# Autodesk Inventor assembly: R2_オムニ
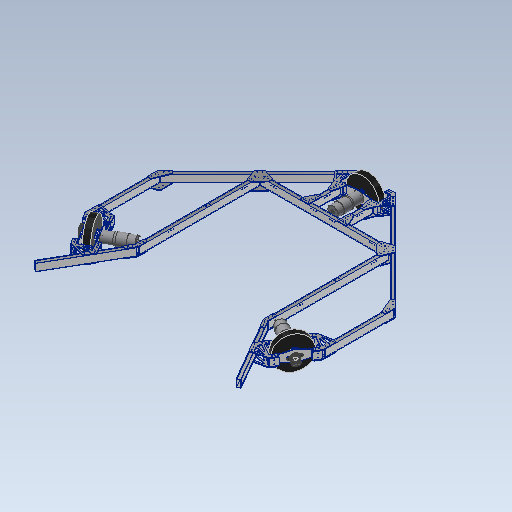
[picture p0: Inventor's stored thumbnail of the model, 512x512]
Saved by Autodesk Inventor 2021 (Build 250183000, 183)
## iProperties
Created: 2021-12-02
Part Number: R2_オムニ
Material: 一般
Document SubType Name: Assembly
Designer: 堀川皓史
Mass: 8176.66 g
Surface Area: 23070.1 cm^2
Volume: 4150.36 cm^3
Density: 1.97011 g/cm^3
Author: 堀川皓史
## Documents named in this file (23)
- C:\Users\hirohumi\OneDrive\ドキュメント\ロボ研\2022NHKロボコン\R2_version1\R2_オムニ.iam
- C:\Users\hirohumi\OneDrive\ドキュメント\ロボ研\2022NHKロボコン\オムニホイール\角柱40mm_モータエンコーダ固定用.ipt
- C:\Users\hirohumi\OneDrive\ドキュメント\ロボ研\2022NHKロボコン\オムニホイール\ホイールユニット_モータ固定板.ipt
- C:\Users\hirohumi\OneDrive\ドキュメント\ロボ研\2022NHKロボコン\オムニホイール\RS-775GM017 v1.ipt
- C:\Users\hirohumi\OneDrive\ドキュメント\ロボ研\2022NHKロボコン\オムニホイール\ホイールユニット_エンコーダ取付板.ipt
- C:\Users\hirohumi\OneDrive\ドキュメント\ロボ研\2022NHKロボコン\オムニホイール\amt102-v v3\amt102-v.iam
- C:\Users\hirohumi\OneDrive\ドキュメント\ロボ研\2022NHKロボコン\オムニホイール\オムニホイール_8-135.ipt
- C:\Users\hirohumi\OneDrive\ドキュメント\ロボ研\2022NHKロボコン\オムニホイール\オムニ固定する.ipt
- C:\Users\hirohumi\OneDrive\ドキュメント\ロボ研\2022NHKロボコン\R2_version1\オムニ_後ろ側板.ipt
- C:\Users\hirohumi\OneDrive\ドキュメント\ロボ研\2022NHKロボコン\R2_version1\オムニ_前1側板.ipt
- C:\Users\hirohumi\OneDrive\ドキュメント\ロボ研\2022NHKロボコン\R2_version1\オムニ_前2側板.ipt
- C:\Users\hirohumi\OneDrive\ドキュメント\ロボ研\2022NHKロボコン\R2_version1\オムニ_角柱1.ipt
- C:\Users\hirohumi\OneDrive\ドキュメント\ロボ研\2022NHKロボコン\オムニホイール\角柱40mm_モータエンコーダ固定用小.ipt
- C:\Users\hirohumi\OneDrive\ドキュメント\ロボ研\2022NHKロボコン\R2_version1\オムニ_固定具1.ipt
- C:\Users\hirohumi\OneDrive\ドキュメント\ロボ研\2022NHKロボコン\R2_version1\オムニ_角柱2.ipt
- C:\Users\hirohumi\OneDrive\ドキュメント\ロボ研\2022NHKロボコン\R2_version1\オムニ_角柱5.ipt
- C:\Users\hirohumi\OneDrive\ドキュメント\ロボ研\2022NHKロボコン\R2_version1\オムニ_固定具2.ipt
- C:\Users\hirohumi\OneDrive\ドキュメント\ロボ研\2022NHKロボコン\R2_version1\オムニ_角柱3.ipt
- C:\Users\hirohumi\OneDrive\ドキュメント\ロボ研\2022NHKロボコン\R2_version1\オムニ_角柱4.ipt
- C:\Users\hirohumi\OneDrive\ドキュメント\ロボ研\2022NHKロボコン\R2_version1\オムニ_固定具3.ipt
- C:\Users\hirohumi\OneDrive\ドキュメント\ロボ研\2022NHKロボコン\R2_version1\オムニ_固定具1-1.ipt
- C:\Users\hirohumi\OneDrive\ドキュメント\ロボ研\2022NHKロボコン\R2_version1\オムニ_角柱7.ipt
- C:\Users\hirohumi\OneDrive\ドキュメント\ロボ研\2022NHKロボコン\R2_version1\オムニ_koteigu.ipt
## Components (70 placed, 22 different names)
1. 角柱40mm_モータエンコーダ固定用:1 — 挿入:17, 挿入:18, 挿入:19
2. 角柱40mm_モータエンコーダ固定用:3 — 挿入:21, 挿入:23
3. ホイールユニット_モータ固定板:1
4. RS-775GM017 v1:1
5. ホイールユニット_エンコーダ取付板:1
6. amt102-v:1 [sub-assembly]
7. オムニホイール_8-135:1
8. オムニ固定する:1
9. オムニ固定する:2
10. オムニ_後ろ側板:1 — 挿入:17, 挿入:18, 挿入:77, 挿入:78, 挿入:81, 挿入:82, 挿入:184, 挿入:185
11. オムニ_後ろ側板:2 — 挿入:19
12. オムニ_後ろ側板:3 — 挿入:21
13. オムニ_後ろ側板:4 — 挿入:23, 挿入:79, 挿入:80, 挿入:83, 挿入:84, 挿入:182, 挿入:183
14. 角柱40mm_モータエンコーダ固定用:5 — 挿入:48, 挿入:50, 挿入:111
15. 角柱40mm_モータエンコーダ固定用:7 — 挿入:41, 挿入:42, 挿入:45, 挿入:112
16. ホイールユニット_モータ固定板:2
17. RS-775GM017 v1:2
18. ホイールユニット_エンコーダ取付板:2 — 挿入:95, 挿入:96
19. amt102-v:2 [sub-assembly]
20. オムニホイール_8-135:2
21. オムニ固定する:3
22. オムニ固定する:4
23. オムニ_前2側板:1 — 挿入:41, 挿入:42, 挿入:87, 挿入:88, 挿入:118, 挿入:119
24. オムニ_前2側板:2 — 挿入:45, 挿入:112
25. オムニ_前1側板:1 — 挿入:50, 挿入:85, 挿入:86, 挿入:109, 挿入:110, 挿入:111
26. オムニ_前1側板:2 — 挿入:48, 挿入:150
27. 角柱40mm_モータエンコーダ固定用:9 — 挿入:115, 挿入:116
28. 角柱40mm_モータエンコーダ固定用:11 — 挿入:117
29. ホイールユニット_モータ固定板:3
30. RS-775GM017 v1:3
31. ホイールユニット_エンコーダ取付板:3 — 挿入:93, 挿入:94
32. amt102-v:3 [sub-assembly]
33. オムニホイール_8-135:3
34. オムニ固定する:5
35. オムニ固定する:6
36. オムニ_前2側板:3 — 挿入:91, 挿入:92
37. オムニ_前2側板:4 — 挿入:117, 挿入:120, 挿入:121
38. オムニ_前1側板:3 — 挿入:89, 挿入:90, 挿入:113, 挿入:114, 挿入:116
39. オムニ_前1側板:4 — 挿入:115
40. オムニ_角柱1:1 — 挿入:77, 挿入:78, 挿入:134, 挿入:135, 挿入:144, 挿入:165, 挿入:167
41. オムニ_角柱1:2 — 挿入:79, 挿入:80, 挿入:140, 挿入:141, 挿入:147, 挿入:178, 挿入:181
42. 角柱40mm_モータエンコーダ固定用小:1 — 挿入:81, 挿入:82
43. 角柱40mm_モータエンコーダ固定用小:2 — 挿入:83, 挿入:84
44. 角柱40mm_モータエンコーダ固定用小:3 — 挿入:89, 挿入:90
45. 角柱40mm_モータエンコーダ固定用小:4 — 挿入:85, 挿入:86, 挿入:150
46. 角柱40mm_モータエンコーダ固定用小:5 — 挿入:91, 挿入:92, 挿入:93, 挿入:94
47. 角柱40mm_モータエンコーダ固定用小:6 — 挿入:87, 挿入:88, 挿入:95, 挿入:96
48. オムニ_固定具1:1 — 挿入:164, 挿入:165
49. オムニ_固定具1:2 — 挿入:177, 挿入:178, 挿入:179
50. オムニ_角柱2:1 — 挿入:109, 挿入:110, 挿入:164, 挿入:166
51. オムニ_角柱2:2 — 挿入:113, 挿入:114, 挿入:177, 挿入:179, 挿入:180
52. オムニ_角柱5:1 — 挿入:118, 挿入:119, 挿入:122, 挿入:123, 挿入:124, 挿入:125
53. オムニ_角柱5:2 — 挿入:120, 挿入:121, 挿入:126, 挿入:127, 挿入:128, 挿入:129
54. オムニ_固定具2:1 — 挿入:122, 挿入:123, 挿入:130, 挿入:131
55. オムニ_固定具2:2 — 挿入:124, 挿入:125
56. オムニ_固定具2:3 — 挿入:128, 挿入:129, 挿入:132, 挿入:133
57. オムニ_固定具2:4 — 挿入:126, 挿入:127
58. オムニ_角柱3:1 — 挿入:130, 挿入:131, 挿入:136, 挿入:137, 挿入:145
59. オムニ_角柱3:2 — 挿入:132, 挿入:133, 挿入:143, 挿入:148
60. オムニ_角柱4:1 — 挿入:138, 挿入:139, 挿入:142, 挿入:146, 挿入:149, フラッシュ:1, フラッシュ:2, 挿入:186
61. オムニ_固定具3:1 — 挿入:134, 挿入:135, 挿入:136, 挿入:137, 挿入:138, 挿入:139
62. オムニ_固定具3:2 — 挿入:147, 挿入:148, 挿入:149
63. オムニ_固定具3:3 — 挿入:144, 挿入:145, 挿入:146
64. オムニ_固定具3:4 — 挿入:140, 挿入:141, 挿入:142, 挿入:143
65. オムニ_固定具1-1:1 — 挿入:180, 挿入:181
66. オムニ_固定具1-1:2 — 挿入:166, 挿入:167
67. オムニ_角柱7:1 — 挿入:182, 挿入:183, 挿入:187
68. オムニ_角柱7:2 — 挿入:184, 挿入:185
69. オムニ_koteigu:1 — フラッシュ:1, フラッシュ:2
70. オムニ_koteigu:2 — 挿入:186, 挿入:187
## Relationships (133: Insert 125, Mate 6, Flush 2)
- [Insert]: 角柱40mm_モータエンコーダ固定用:1 ↔ ホイールユニット_モータ固定板:1
- [Insert]: 角柱40mm_モータエンコーダ固定用:1 ↔ ホイールユニット_モータ固定板:1
- [Insert]: 角柱40mm_モータエンコーダ固定用:3 ↔ ホイールユニット_モータ固定板:1
- [Insert]: 角柱40mm_モータエンコーダ固定用:3 ↔ ホイールユニット_モータ固定板:1
- [Insert]: ホイールユニット_モータ固定板:1 ↔ RS-775GM017 v1:1
- [Insert]: ホイールユニット_モータ固定板:1 ↔ RS-775GM017 v1:1
- [Insert]: ホイールユニット_エンコーダ取付板:1 ↔ amt102-v:1
- [Insert]: オムニホイール_8-135:1 ↔ オムニ固定する:1
- [Insert]: オムニホイール_8-135:1 ↔ オムニ固定する:1
- [Insert]: オムニホイール_8-135:1 ↔ オムニ固定する:2
- [Insert]: オムニホイール_8-135:1 ↔ オムニ固定する:2
- [Mate]: RS-775GM017 v1:1 ↔ オムニ固定する:1
- [Mate] (6 mm): ホイールユニット_モータ固定板:1 ↔ オムニ固定する:1
- 挿入:17 [Insert]: 角柱40mm_モータエンコーダ固定用:1 ↔ オムニ_後ろ側板:1
- 挿入:18 [Insert]: 角柱40mm_モータエンコーダ固定用:1 ↔ オムニ_後ろ側板:1
- 挿入:19 [Insert]: 角柱40mm_モータエンコーダ固定用:1 ↔ オムニ_後ろ側板:2
- 挿入:21 [Insert]: 角柱40mm_モータエンコーダ固定用:3 ↔ オムニ_後ろ側板:3
- 挿入:23 [Insert]: 角柱40mm_モータエンコーダ固定用:3 ↔ オムニ_後ろ側板:4
- [Insert]: 角柱40mm_モータエンコーダ固定用:5 ↔ ホイールユニット_モータ固定板:2
- [Insert]: 角柱40mm_モータエンコーダ固定用:5 ↔ ホイールユニット_モータ固定板:2
- [Insert]: 角柱40mm_モータエンコーダ固定用:7 ↔ ホイールユニット_モータ固定板:2
- [Insert]: 角柱40mm_モータエンコーダ固定用:7 ↔ ホイールユニット_モータ固定板:2
- [Insert]: ホイールユニット_モータ固定板:2 ↔ RS-775GM017 v1:2
- [Insert]: ホイールユニット_モータ固定板:2 ↔ RS-775GM017 v1:2
- [Insert]: ホイールユニット_エンコーダ取付板:2 ↔ amt102-v:2
- [Insert]: オムニホイール_8-135:2 ↔ オムニ固定する:3
- [Insert]: オムニホイール_8-135:2 ↔ オムニ固定する:3
- [Insert]: オムニホイール_8-135:2 ↔ オムニ固定する:4
- [Insert]: オムニホイール_8-135:2 ↔ オムニ固定する:4
- [Mate]: RS-775GM017 v1:2 ↔ オムニ固定する:3
- [Mate] (6 mm): ホイールユニット_モータ固定板:2 ↔ オムニ固定する:3
- 挿入:41 [Insert]: 角柱40mm_モータエンコーダ固定用:7 ↔ オムニ_前2側板:1
- 挿入:42 [Insert]: 角柱40mm_モータエンコーダ固定用:7 ↔ オムニ_前2側板:1
- 挿入:45 [Insert]: 角柱40mm_モータエンコーダ固定用:7 ↔ オムニ_前2側板:2
- 挿入:48 [Insert]: 角柱40mm_モータエンコーダ固定用:5 ↔ オムニ_前1側板:2
- 挿入:50 [Insert]: 角柱40mm_モータエンコーダ固定用:5 ↔ オムニ_前1側板:1
- [Insert]: 角柱40mm_モータエンコーダ固定用:9 ↔ ホイールユニット_モータ固定板:3
- [Insert]: 角柱40mm_モータエンコーダ固定用:9 ↔ ホイールユニット_モータ固定板:3
- [Insert]: 角柱40mm_モータエンコーダ固定用:11 ↔ ホイールユニット_モータ固定板:3
- [Insert]: 角柱40mm_モータエンコーダ固定用:11 ↔ ホイールユニット_モータ固定板:3
- [Insert]: ホイールユニット_モータ固定板:3 ↔ RS-775GM017 v1:3
- [Insert]: ホイールユニット_モータ固定板:3 ↔ RS-775GM017 v1:3
- [Insert]: ホイールユニット_エンコーダ取付板:3 ↔ amt102-v:3
- [Insert]: オムニホイール_8-135:3 ↔ オムニ固定する:5
- [Insert]: オムニホイール_8-135:3 ↔ オムニ固定する:5
- [Insert]: オムニホイール_8-135:3 ↔ オムニ固定する:6
- [Insert]: オムニホイール_8-135:3 ↔ オムニ固定する:6
- [Mate]: RS-775GM017 v1:3 ↔ オムニ固定する:5
- [Mate] (6 mm): ホイールユニット_モータ固定板:3 ↔ オムニ固定する:5
- [Insert]: 角柱40mm_モータエンコーダ固定用:11 ↔ オムニ_前2側板:3
- [Insert]: 角柱40mm_モータエンコーダ固定用:11 ↔ オムニ_前2側板:3
- [Insert]: 角柱40mm_モータエンコーダ固定用:11 ↔ オムニ_前2側板:4
- [Insert]: 角柱40mm_モータエンコーダ固定用:9 ↔ オムニ_前1側板:4
- [Insert]: 角柱40mm_モータエンコーダ固定用:9 ↔ オムニ_前1側板:3
- 挿入:77 [Insert]: オムニ_後ろ側板:1 ↔ オムニ_角柱1:1
- 挿入:78 [Insert]: オムニ_後ろ側板:1 ↔ オムニ_角柱1:1
- 挿入:79 [Insert]: オムニ_後ろ側板:4 ↔ オムニ_角柱1:2
- 挿入:80 [Insert]: オムニ_後ろ側板:4 ↔ オムニ_角柱1:2
- 挿入:81 [Insert]: オムニ_後ろ側板:1 ↔ 角柱40mm_モータエンコーダ固定用小:1
- 挿入:82 [Insert]: オムニ_後ろ側板:1 ↔ 角柱40mm_モータエンコーダ固定用小:1
- 挿入:83 [Insert]: オムニ_後ろ側板:4 ↔ 角柱40mm_モータエンコーダ固定用小:2
- 挿入:84 [Insert]: オムニ_後ろ側板:4 ↔ 角柱40mm_モータエンコーダ固定用小:2
- 挿入:85 [Insert]: オムニ_前1側板:1 ↔ 角柱40mm_モータエンコーダ固定用小:4
- 挿入:86 [Insert]: オムニ_前1側板:1 ↔ 角柱40mm_モータエンコーダ固定用小:4
- 挿入:87 [Insert]: オムニ_前2側板:1 ↔ 角柱40mm_モータエンコーダ固定用小:6
- 挿入:88 [Insert]: オムニ_前2側板:1 ↔ 角柱40mm_モータエンコーダ固定用小:6
- 挿入:89 [Insert]: オムニ_前1側板:3 ↔ 角柱40mm_モータエンコーダ固定用小:3
- 挿入:90 [Insert]: オムニ_前1側板:3 ↔ 角柱40mm_モータエンコーダ固定用小:3
- 挿入:91 [Insert]: オムニ_前2側板:3 ↔ 角柱40mm_モータエンコーダ固定用小:5
- 挿入:92 [Insert]: オムニ_前2側板:3 ↔ 角柱40mm_モータエンコーダ固定用小:5
- 挿入:93 [Insert]: ホイールユニット_エンコーダ取付板:3 ↔ 角柱40mm_モータエンコーダ固定用小:5
- 挿入:94 [Insert]: ホイールユニット_エンコーダ取付板:3 ↔ 角柱40mm_モータエンコーダ固定用小:5
- 挿入:95 [Insert]: ホイールユニット_エンコーダ取付板:2 ↔ 角柱40mm_モータエンコーダ固定用小:6
- 挿入:96 [Insert]: ホイールユニット_エンコーダ取付板:2 ↔ 角柱40mm_モータエンコーダ固定用小:6
- 挿入:109 [Insert]: オムニ_前1側板:1 ↔ オムニ_角柱2:1
- 挿入:110 [Insert]: オムニ_前1側板:1 ↔ オムニ_角柱2:1
- 挿入:111 [Insert]: 角柱40mm_モータエンコーダ固定用:5 ↔ オムニ_前1側板:1
- 挿入:112 [Insert]: 角柱40mm_モータエンコーダ固定用:7 ↔ オムニ_前2側板:2
- 挿入:113 [Insert]: オムニ_前1側板:3 ↔ オムニ_角柱2:2
- 挿入:114 [Insert]: オムニ_前1側板:3 ↔ オムニ_角柱2:2
- 挿入:115 [Insert]: 角柱40mm_モータエンコーダ固定用:9 ↔ オムニ_前1側板:4
- 挿入:116 [Insert]: 角柱40mm_モータエンコーダ固定用:9 ↔ オムニ_前1側板:3
- 挿入:117 [Insert]: 角柱40mm_モータエンコーダ固定用:11 ↔ オムニ_前2側板:4
- 挿入:118 [Insert]: オムニ_前2側板:1 ↔ オムニ_角柱5:1
- 挿入:119 [Insert]: オムニ_前2側板:1 ↔ オムニ_角柱5:1
- 挿入:120 [Insert]: オムニ_前2側板:4 ↔ オムニ_角柱5:2
- 挿入:121 [Insert]: オムニ_前2側板:4 ↔ オムニ_角柱5:2
- 挿入:122 [Insert]: オムニ_角柱5:1 ↔ オムニ_固定具2:1
- 挿入:123 [Insert]: オムニ_角柱5:1 ↔ オムニ_固定具2:1
- 挿入:124 [Insert]: オムニ_角柱5:1 ↔ オムニ_固定具2:2
- 挿入:125 [Insert]: オムニ_角柱5:1 ↔ オムニ_固定具2:2
- 挿入:126 [Insert]: オムニ_角柱5:2 ↔ オムニ_固定具2:4
- 挿入:127 [Insert]: オムニ_角柱5:2 ↔ オムニ_固定具2:4
- 挿入:128 [Insert]: オムニ_角柱5:2 ↔ オムニ_固定具2:3
- 挿入:129 [Insert]: オムニ_角柱5:2 ↔ オムニ_固定具2:3
- 挿入:130 [Insert]: オムニ_固定具2:1 ↔ オムニ_角柱3:1
- 挿入:131 [Insert]: オムニ_固定具2:1 ↔ オムニ_角柱3:1
- 挿入:132 [Insert]: オムニ_固定具2:3 ↔ オムニ_角柱3:2
- 挿入:133 [Insert]: オムニ_固定具2:3 ↔ オムニ_角柱3:2
- 挿入:134 [Insert]: オムニ_角柱1:1 ↔ オムニ_固定具3:1
- 挿入:135 [Insert]: オムニ_角柱1:1 ↔ オムニ_固定具3:1
- 挿入:136 [Insert]: オムニ_角柱3:1 ↔ オムニ_固定具3:1
- 挿入:137 [Insert]: オムニ_角柱3:1 ↔ オムニ_固定具3:1
- 挿入:138 [Insert]: オムニ_角柱4:1 ↔ オムニ_固定具3:1
- 挿入:139 [Insert]: オムニ_角柱4:1 ↔ オムニ_固定具3:1
- 挿入:140 [Insert]: オムニ_角柱1:2 ↔ オムニ_固定具3:4
- 挿入:141 [Insert]: オムニ_角柱1:2 ↔ オムニ_固定具3:4
- 挿入:142 [Insert]: オムニ_角柱4:1 ↔ オムニ_固定具3:4
- 挿入:143 [Insert]: オムニ_角柱3:2 ↔ オムニ_固定具3:4
- 挿入:144 [Insert]: オムニ_角柱1:1 ↔ オムニ_固定具3:3
- 挿入:145 [Insert]: オムニ_角柱3:1 ↔ オムニ_固定具3:3
- 挿入:146 [Insert]: オムニ_角柱4:1 ↔ オムニ_固定具3:3
- 挿入:147 [Insert]: オムニ_角柱1:2 ↔ オムニ_固定具3:2
- 挿入:148 [Insert]: オムニ_角柱3:2 ↔ オムニ_固定具3:2
- 挿入:149 [Insert]: オムニ_角柱4:1 ↔ オムニ_固定具3:2
- 挿入:150 [Insert]: オムニ_前1側板:2 ↔ 角柱40mm_モータエンコーダ固定用小:4
- 挿入:164 [Insert]: オムニ_固定具1:1 ↔ オムニ_角柱2:1
- 挿入:165 [Insert]: オムニ_角柱1:1 ↔ オムニ_固定具1:1
- 挿入:166 [Insert]: オムニ_角柱2:1 ↔ オムニ_固定具1-1:2
- 挿入:167 [Insert]: オムニ_角柱1:1 ↔ オムニ_固定具1-1:2
- 挿入:177 [Insert]: オムニ_固定具1:2 ↔ オムニ_角柱2:2
- 挿入:178 [Insert]: オムニ_角柱1:2 ↔ オムニ_固定具1:2
- 挿入:179 [Insert]: オムニ_固定具1:2 ↔ オムニ_角柱2:2
- 挿入:180 [Insert]: オムニ_角柱2:2 ↔ オムニ_固定具1-1:1
- 挿入:181 [Insert]: オムニ_角柱1:2 ↔ オムニ_固定具1-1:1
- 挿入:182 [Insert]: オムニ_後ろ側板:4 ↔ オムニ_角柱7:1
- 挿入:183 [Insert]: オムニ_後ろ側板:4 ↔ オムニ_角柱7:1
- 挿入:184 [Insert]: オムニ_後ろ側板:1 ↔ オムニ_角柱7:2
- 挿入:185 [Insert]: オムニ_後ろ側板:1 ↔ オムニ_角柱7:2
- フラッシュ:1 [Flush]: オムニ_角柱4:1 ↔ オムニ_koteigu:1
- フラッシュ:2 [Flush]: オムニ_角柱4:1 ↔ オムニ_koteigu:1
- 挿入:186 [Insert]: オムニ_角柱4:1 ↔ オムニ_koteigu:2
- 挿入:187 [Insert]: オムニ_角柱7:1 ↔ オムニ_koteigu:2
## Named parameters: d41_d93 = 6 mm, d42_d30 = 0 mm, d43_d31 = 0 mm, d44_d32 = 0 mm, d45_d33 = 0 mm, d46_d34 = 0 mm, d47_d16 = 0 mm, d48_d17 = 0 mm, d49_d18 = 0 mm, d50_d19 = 0 mm, d51_d24 = 0 mm, d52_d25 = 0 mm, d56_d29 = 0 mm, d69_d63 = 0 mm, d72_d66 = 0 mm, d74_d68 = 0 mm, d77_d59 = 0 mm, d78_d60 = 0 mm, d81_d41_d93 = 6 mm, d82_d42_d30 = 0 mm, d83_d43_d31 = 0 mm, d84_d44_d32 = 0 mm, d85_d45_d33 = 0 mm, d86_d46_d34 = 0 mm, d87_d47_d16 = 0 mm, d88_d48_d17 = 0 mm, d89_d49_d18 = 0 mm, d90_d50_d19 = 0 mm, d91_d51_d24 = 0 mm, d92_d52_d25 = 0 mm, d97_d56_d29 = 0 mm
